# Autodesk Inventor assembly: RobLink2
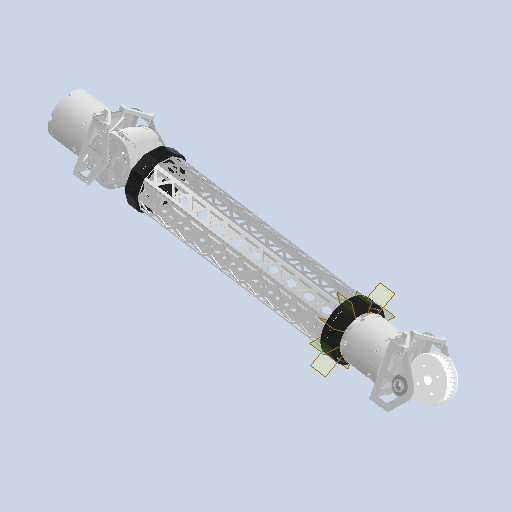
[picture p0: Inventor's stored thumbnail of the model, 512x512]
Saved by Autodesk Inventor 2024 (Build 280153000, 153)
## iProperties
Created: 2025-02-08
Part Number: RobLink2
Document SubType Name: Assembly
Designer: tanoue_kota
Mass: 1315.61 g
Surface Area: 3333.08 cm^2
Volume: 281.501 cm^3
Density: 4.67356 g/cm^3
Author: tanoue_kota
## Documents named in this file (22)
- C:\Users\田之上巧太\Documents\Inventor\RobArm\rob_link2\RobLink2.iam
- C:\Users\田之上巧太\Documents\Inventor\RobArm\rob_link2\roblink2_parameter.ipt
- C:\Users\田之上巧太\Documents\Inventor\RobArm\Actuator\RS00\RS00.iam
- C:\Users\田之上巧太\Documents\Inventor\RobArm\rob_link2\link2plate1.ipt
- C:\Users\田之上巧太\Documents\Inventor\RobArm\rob_link2\link2part1.ipt
- C:\Users\田之上巧太\Documents\Inventor\RobArm\rob_link2\link2plate2.ipt
- C:\Users\田之上巧太\Documents\Inventor\RobArm\rob_link2\link2part2.ipt
- C:\Users\田之上巧太\Documents\Inventor\RobArm\rob_link2\link2part4.ipt
- C:\Users\田之上巧太\Documents\Inventor\RobArm\rob_link2\link2plate3.ipt
- C:\Users\田之上巧太\Documents\Inventor\RobArm\rob_link2\link2plate4.ipt
- C:\Users\田之上巧太\Documents\Inventor\RobArm\rob_link2\link2part5.ipt
- C:\Users\田之上巧太\Documents\Inventor\RobArm\BasicParts\Bearing\FL6800ZZ.ipt
- C:\Users\田之上巧太\Documents\Inventor\RobArm\rob_link2\link2plate5.ipt
- C:\Users\田之上巧太\Documents\Inventor\RobArm\rob_link2\link2part6.ipt
- C:\Users\田之上巧太\Documents\Inventor\RobArm\rob_link2\link2part7.ipt
- C:\Users\田之上巧太\Documents\Inventor\RobArm\rob_link2\link2part8.ipt
- C:\Users\田之上巧太\Documents\Inventor\RobArm\rob_link1\link1plate6.ipt
- C:\Users\田之上巧太\Documents\Inventor\RobArm\rob_link2\timingpulley2.ipt
- C:\Users\田之上巧太\Documents\Inventor\RobArm\BasicParts\Bearing\C-SFL678ZZ_STEP_AP203_20250215\C-SFL678ZZ\C-SFL678ZZ.ipt
- C:\Users\田之上巧太\Documents\Inventor\RobArm\rob_link2\link2part9.ipt
- C:\Users\田之上巧太\Documents\Inventor\RobArm\rob_link2\link2part10.ipt
- C:\Users\田之上巧太\Documents\Inventor\RobArm\rob_link2\link2part10_MIR.ipt
## Components (27 placed, 21 different names)
1. roblink2_parameter:1
2. RS00:1 [sub-assembly] — 回転:19, メイト:1, 回転:54, 回転:55
3. link2plate1:1 — 回転:1, 回転:20, 回転:21, 回転:23, 回転:24, 回転:25, 回転:43, 回転:44, 回転:51, 回転:52, 回転:53, 回転:58, 回転:59, 回転:60
4. link2part1:1 — 回転:45, 回転:46, 回転:58, 回転:59
5. link2plate2:1 — 回転:1, 回転:60
6. link2part2:1 — 回転:19, メイト:1, 回転:45, 回転:46
7. link2part4:1 — 回転:20, 回転:21, 回転:33, 回転:47, 回転:51, 回転:52
8. link2part4:2 — 回転:23, 回転:30, 回転:50, 回転:53
9. RS00:2 [sub-assembly] — 回転:28, 回転:29, 回転:34, 回転:35, 回転:48, 回転:49
10. link2plate3:1 — 回転:28, 回転:29, 回転:33, 回転:47, 回転:65, 回転:66
11. link2plate4:1 — 回転:30, 回転:48, 回転:49, 回転:50, メイト:16, メイト:17, 回転:63, 回転:64
12. link2part5:1 — 回転:24, 回転:25, 回転:43, 回転:44, 回転:63, 回転:64, 回転:65, 回転:66
13. link2plate5:1 — 回転:36, メイト:4, 回転:37, メイト:5, メイト:6, メイト:7, メイト:8, メイト:9, メイト:10, 回転:38, 回転:39, メイト:11
14. link2part6:1 — 回転:34, 回転:35, 回転:36, メイト:4, メイト:11
15. link2part7:1 — 回転:37
16. link2part8:1 — メイト:5, メイト:6, メイト:7
17. link2part8:2 — メイト:8, メイト:9, メイト:10
18. RS00:3 [sub-assembly] — 回転:38, 回転:39
19. link1plate6:1 — 回転:54, 回転:55, メイト:12, メイト:13, メイト:14, メイト:15, 回転:56, 回転:57, メイト:18, メイト:19, メイト:20, メイト:21, メイト:22, メイト:23
20. FL6800ZZ:2 — メイト:12, メイト:13, 回転:62
21. FL6800ZZ:3 — メイト:14, メイト:15, 回転:61
22. timingpulley2:1 — 回転:56, 回転:57
23. C-SFL678ZZ:1 — メイト:16, メイト:17
24. link2part9:1 — 回転:61
25. link2part9:2 — 回転:62
26. link2part10:1 — メイト:18, メイト:19, メイト:20
27. link2part10_MIR:1 — メイト:21, メイト:22, メイト:23
## Relationships (62: RevoluteJoint 41, Mate 21)
- 回転:1 [RevoluteJoint]: link2plate1:1 ↔ link2plate2:1
- 回転:19 [RevoluteJoint]: RS00:1 ↔ link2part2:1
- メイト:1 [Mate]: RS00:1 ↔ link2part2:1
- 回転:20 [RevoluteJoint]: link2plate1:1 ↔ link2part4:1
- 回転:21 [RevoluteJoint]: link2plate1:1 ↔ link2part4:1
- 回転:23 [RevoluteJoint]: link2plate1:1 ↔ link2part4:2
- 回転:24 [RevoluteJoint]: link2plate1:1 ↔ link2part5:1
- 回転:25 [RevoluteJoint]: link2plate1:1 ↔ link2part5:1
- 回転:28 [RevoluteJoint]: RS00:2 ↔ link2plate3:1
- 回転:29 [RevoluteJoint]: RS00:2 ↔ link2plate3:1
- 回転:30 [RevoluteJoint]: link2part4:2 ↔ link2plate4:1
- 回転:33 [RevoluteJoint]: link2part4:1 ↔ link2plate3:1
- 回転:34 [RevoluteJoint]: RS00:2 ↔ link2part6:1
- 回転:35 [RevoluteJoint]: RS00:2 ↔ link2part6:1
- 回転:36 [RevoluteJoint]: link2plate5:1 ↔ link2part6:1
- メイト:4 [Mate]: link2plate5:1 ↔ link2part6:1
- 回転:37 [RevoluteJoint]: link2plate5:1 ↔ link2part7:1
- メイト:5 [Mate]: link2plate5:1 ↔ link2part8:1
- メイト:6 [Mate]: link2plate5:1 ↔ link2part8:1
- メイト:7 [Mate]: link2plate5:1 ↔ link2part8:1
- メイト:8 [Mate]: link2plate5:1 ↔ link2part8:2
- メイト:9 [Mate]: link2plate5:1 ↔ link2part8:2
- メイト:10 [Mate]: link2plate5:1 ↔ link2part8:2
- 回転:38 [RevoluteJoint]: link2plate5:1 ↔ RS00:3
- 回転:39 [RevoluteJoint]: link2plate5:1 ↔ RS00:3
- メイト:11 [Mate]: link2plate5:1 ↔ link2part6:1
- 回転:43 [RevoluteJoint]: link2plate1:1 ↔ link2part5:1
- 回転:44 [RevoluteJoint]: link2plate1:1 ↔ link2part5:1
- 回転:45 [RevoluteJoint]: link2part1:1 ↔ link2part2:1
- 回転:46 [RevoluteJoint]: link2part1:1 ↔ link2part2:1
- 回転:47 [RevoluteJoint]: link2part4:1 ↔ link2plate3:1
- 回転:48 [RevoluteJoint]: RS00:2 ↔ link2plate4:1
- 回転:49 [RevoluteJoint]: RS00:2 ↔ link2plate4:1
- 回転:50 [RevoluteJoint]: link2part4:2 ↔ link2plate4:1
- 回転:51 [RevoluteJoint]: link2plate1:1 ↔ link2part4:1
- 回転:52 [RevoluteJoint]: link2plate1:1 ↔ link2part4:1
- 回転:53 [RevoluteJoint]: link2plate1:1 ↔ link2part4:2
- 回転:54 [RevoluteJoint]: RS00:1 ↔ link1plate6:1
- 回転:55 [RevoluteJoint]: RS00:1 ↔ link1plate6:1
- メイト:12 [Mate]: link1plate6:1 ↔ FL6800ZZ:2
- メイト:13 [Mate]: link1plate6:1 ↔ FL6800ZZ:2
- メイト:14 [Mate]: link1plate6:1 ↔ FL6800ZZ:3
- メイト:15 [Mate]: link1plate6:1 ↔ FL6800ZZ:3
- 回転:56 [RevoluteJoint]: link1plate6:1 ↔ timingpulley2:1
- 回転:57 [RevoluteJoint]: link1plate6:1 ↔ timingpulley2:1
- メイト:16 [Mate]: link2plate4:1 ↔ C-SFL678ZZ:1
- メイト:17 [Mate]: link2plate4:1 ↔ C-SFL678ZZ:1
- 回転:58 [RevoluteJoint]: link2plate1:1 ↔ link2part1:1
- 回転:59 [RevoluteJoint]: link2plate1:1 ↔ link2part1:1
- 回転:60 [RevoluteJoint]: link2plate1:1 ↔ link2plate2:1
- 回転:61 [RevoluteJoint]: FL6800ZZ:3 ↔ link2part9:1
- 回転:62 [RevoluteJoint]: FL6800ZZ:2 ↔ link2part9:2
- 回転:63 [RevoluteJoint]: link2plate4:1 ↔ link2part5:1
- 回転:64 [RevoluteJoint]: link2plate4:1 ↔ link2part5:1
- 回転:65 [RevoluteJoint]: link2plate3:1 ↔ link2part5:1
- 回転:66 [RevoluteJoint]: link2plate3:1 ↔ link2part5:1
- メイト:18 [Mate]: link1plate6:1 ↔ link2part10:1
- メイト:19 [Mate]: link1plate6:1 ↔ link2part10:1
- メイト:20 [Mate]: link1plate6:1 ↔ link2part10:1
- メイト:21 [Mate]: link1plate6:1 ↔ link2part10_MIR:1
- メイト:22 [Mate]: link1plate6:1 ↔ link2part10_MIR:1
- メイト:23 [Mate]: link1plate6:1 ↔ link2part10_MIR:1
